# Autodesk Inventor assembly: 2022Drivetrain-v1
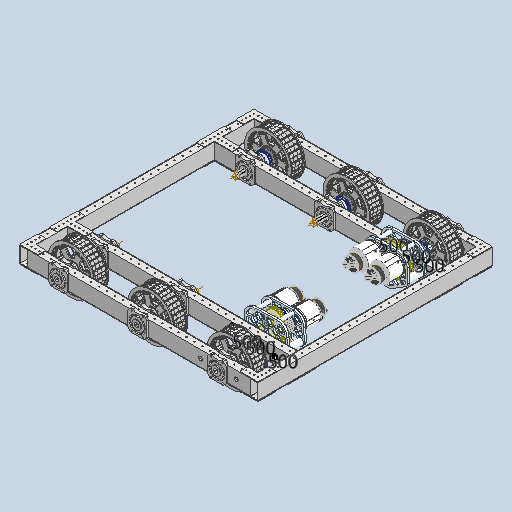
[picture p0: Inventor's stored thumbnail of the model, 512x512]
Saved by Autodesk Inventor 2022 (Build 260153000, 153)
## iProperties
Created: 2022-01-09
Part Number: 2022Drivetrain-v1
Document SubType Name: Assembly
Designer: merky
Author: merky
## Documents named in this file (11)
- C:\Users\tagaz\OneDrive\Documents\T3-Cad\CAD\2022 Parts\Drivetrain\2022Drivetrain-v1.iam
- C:\Users\tagaz\OneDrive\Documents\T3-Cad\CAD\2022 Parts\Generic\VersaFrame 28in.ipt
- C:\Users\tagaz\OneDrive\Documents\T3-Cad\CAD\2022 Parts\Generic\VersaFrame 30in.ipt
- C:\Users\tagaz\OneDrive\Documents\T3-Cad\CAD\VersaBlock Assembly.iam
- C:\Users\tagaz\OneDrive\Documents\T3-Cad\CAD\2022 Parts\Generic\VersaBlock Assemblyv2.iam
- C:\Users\tagaz\OneDrive\Documents\T3-Cad\CAD\Traction Wheel Assembly.iam
- C:\Users\tagaz\OneDrive\Documents\T3-Cad\CAD\6in x 1.5in Wheel.iam
- C:\Users\tagaz\OneDrive\Documents\T3-Cad\CAD\Generic and Stock\T Gusset.ipt
- C:\Users\tagaz\OneDrive\Documents\T3-Cad\CAD\2022 Parts\Generic\ShortenedVersaGusset 90o.ipt
- C:\Users\tagaz\OneDrive\Documents\T3-Cad\CAD\Generic and Stock\15T Sprocket.ipt
- C:\Users\tagaz\OneDrive\Documents\T3-Cad\CAD\2022 Parts\Generic\NewGearboxAssembly.iam
## Components (40 placed, 10 different names)
1. 15T Sprocket:1 — Insert:11
2. 15T Sprocket:2 — Insert:12
3. VersaFrame 28in:4 — Mate:17, Flush:9, Flush:10, Mate:27, Mate:28, Mate:30, Mate:31, Mate:33, Mate:34, Flush:11, Flush:13, Flush:16, Flush:18
4. VersaFrame 28in:3 — Mate:16, Flush:7, Flush:8, Mate:18, Mate:19, Mate:21, Mate:22, Mate:24, Mate:25, Flush:19, Flush:21, Flush:24, Flush:26
5. VersaFrame 30in:2 — Flush:1, Flush:2, Mate:1, Flush:3, Flush:4, Mate:3, Flush:5, Flush:6, Mate:6, Mate:9, Mate:12, Mate:15, Mate:16, Flush:7, Flush:8, Mate:17, Flush:9, Flush:10, Mate:20, Mate:23, Mate:26, Mate:29, Mate:32, Mate:35, Mate:36, Flush:12, Mate:37, Flush:14, Mate:40, Flush:20, Mate:41, Flush:22, Mate:48, Flush:35, Mate:49, Flush:37, Mate:50, Flush:40, Mate:51, Flush:42
6. VersaFrame 30in:1 — Flush:1, Flush:2, Mate:2, Mate:38, Flush:15, Mate:39, Flush:17, Mate:42, Flush:23, Mate:43, Flush:25, Mate:46, Flush:31, Mate:47, Flush:34
7. VersaFrame 28in:2 — Mate:3, Flush:5, Flush:6, Mate:10, Mate:11, Mate:13, Mate:14, Flush:32, Flush:39, Flush:41, Insert:8
8. VersaFrame 28in:1 — Mate:1, Flush:3, Flush:4, Mate:2, Mate:4, Mate:5, Mate:7, Mate:8, Flush:33, Flush:36, Flush:38, Insert:7
9. NewGearboxAssembly:1 [sub-assembly] — Insert:7, Insert:9, Insert:12
10. VersaBlock Assembly:1 [sub-assembly] — Mate:10, Mate:11, Mate:12, Insert:6
11. VersaBlock Assembly:3 [sub-assembly] — Mate:7, Mate:8, Mate:9, Insert:4
12. VersaBlock Assembly:4 [sub-assembly] — Mate:4, Mate:5, Mate:6, Insert:3
13. VersaBlock Assemblyv2:1 [sub-assembly] — Mate:13, Mate:14, Mate:15, Insert:5
14. Traction Wheel Assembly:1 [sub-assembly] — Insert:3
15. Traction Wheel Assembly:2 [sub-assembly] — Insert:4
16. Traction Wheel Assembly:3 [sub-assembly] — Insert:5
17. Traction Wheel Assembly:4 [sub-assembly] — Insert:6
18. 6in x 1.5in Wheel:1 [sub-assembly] — Insert:10
19. 6in x 1.5in Wheel:2 [sub-assembly] — Insert:9
20. VersaBlock Assembly:5 [sub-assembly] — Mate:18, Mate:19, Mate:20
21. VersaBlock Assembly:6 [sub-assembly] — Mate:21, Mate:22, Mate:23
22. VersaBlock Assembly:7 [sub-assembly] — Mate:24, Mate:25, Mate:26
23. VersaBlock Assembly:8 [sub-assembly] — Mate:33, Mate:34, Mate:35
24. VersaBlock Assembly:9 [sub-assembly] — Mate:30, Mate:31, Mate:32
25. VersaBlock Assembly:10 [sub-assembly] — Mate:27, Mate:28, Mate:29
26. NewGearboxAssembly:2 [sub-assembly] — Insert:8, Insert:10, Insert:11
27. T Gusset:1 — Mate:48, Flush:35, Flush:36
28. T Gusset:2 — Mate:49, Flush:37, Flush:38
29. T Gusset:5 — Mate:46, Flush:31, Flush:32
30. T Gusset:6 — Mate:47, Flush:33, Flush:34
31. T Gusset:7 — Mate:51, Flush:41, Flush:42
32. T Gusset:8 — Mate:50, Flush:39, Flush:40
33. ShortenedVersaGusset 90o:1 — Mate:40, Flush:19, Flush:20
34. ShortenedVersaGusset 90o:2 — Mate:41, Flush:21, Flush:22
35. ShortenedVersaGusset 90o:3 — Mate:37, Flush:13, Flush:14
36. ShortenedVersaGusset 90o:4 — Mate:36, Flush:11, Flush:12
37. ShortenedVersaGusset 90o:5 — Mate:39, Flush:17, Flush:18
38. ShortenedVersaGusset 90o:6 — Mate:38, Flush:15, Flush:16
39. ShortenedVersaGusset 90o:7 — Mate:43, Flush:25, Flush:26
40. ShortenedVersaGusset 90o:8 — Mate:42, Flush:23, Flush:24
## Relationships (97: Mate 49, Flush 38, Insert 10)
- Flush:1: VersaFrame 30in:2 ↔ VersaFrame 30in:1
- Flush:2: VersaFrame 30in:2 ↔ VersaFrame 30in:1
- Mate:1: VersaFrame 30in:2 ↔ VersaFrame 28in:1
- Flush:3: VersaFrame 30in:2 ↔ VersaFrame 28in:1
- Flush:4 (127 mm): VersaFrame 30in:2 ↔ VersaFrame 28in:1
- Mate:2: VersaFrame 30in:1 ↔ VersaFrame 28in:1
- Mate:3: VersaFrame 30in:2 ↔ VersaFrame 28in:2
- Flush:5: VersaFrame 30in:2 ↔ VersaFrame 28in:2
- Flush:6 (127 mm): VersaFrame 30in:2 ↔ VersaFrame 28in:2
- Mate:4: VersaFrame 28in:1 ↔ VersaBlock Assembly:4
- Mate:5: VersaFrame 28in:1 ↔ VersaBlock Assembly:4
- Mate:6 (71.0692 mm): VersaFrame 30in:2 ↔ VersaBlock Assembly:4
- Mate:7: VersaFrame 28in:1 ↔ VersaBlock Assembly:3
- Mate:8: VersaFrame 28in:1 ↔ VersaBlock Assembly:3
- Mate:9 (325.0692 mm): VersaFrame 30in:2 ↔ VersaBlock Assembly:3
- Mate:10: VersaFrame 28in:2 ↔ VersaBlock Assembly:1
- Mate:11: VersaFrame 28in:2 ↔ VersaBlock Assembly:1
- Mate:12 (71.0692 mm): VersaFrame 30in:2 ↔ VersaBlock Assembly:1
- Mate:13: VersaFrame 28in:2 ↔ VersaBlock Assemblyv2:1
- Mate:14: VersaFrame 28in:2 ↔ VersaBlock Assemblyv2:1
- Mate:15 (325.0692 mm): VersaFrame 30in:2 ↔ VersaBlock Assemblyv2:1
- Insert:3 (-63.5 mm): VersaBlock Assembly:4 ↔ Traction Wheel Assembly:1
- Insert:4 (-63.5 mm): VersaBlock Assembly:3 ↔ Traction Wheel Assembly:2
- Mate:16: VersaFrame 28in:3 ↔ VersaFrame 30in:2
- Flush:7: VersaFrame 28in:3 ↔ VersaFrame 30in:2
- Flush:8: VersaFrame 28in:3 ↔ VersaFrame 30in:2
- Mate:17: VersaFrame 28in:4 ↔ VersaFrame 30in:2
- Flush:9: VersaFrame 28in:4 ↔ VersaFrame 30in:2
- Flush:10: VersaFrame 28in:4 ↔ VersaFrame 30in:2
- Insert:5 (-63.5 mm): VersaBlock Assemblyv2:1 ↔ Traction Wheel Assembly:3
- Insert:6 (-63.5 mm): VersaBlock Assembly:1 ↔ Traction Wheel Assembly:4
- Mate:18: VersaFrame 28in:3 ↔ VersaBlock Assembly:5
- Mate:19: VersaFrame 28in:3 ↔ VersaBlock Assembly:5
- Mate:20 (71.0692 mm): VersaFrame 30in:2 ↔ VersaBlock Assembly:5
- Mate:21: VersaFrame 28in:3 ↔ VersaBlock Assembly:6
- Mate:22: VersaFrame 28in:3 ↔ VersaBlock Assembly:6
- Mate:23 (325.0692 mm): VersaFrame 30in:2 ↔ VersaBlock Assembly:6
- Mate:24: VersaFrame 28in:3 ↔ VersaBlock Assembly:7
- Mate:25: VersaFrame 28in:3 ↔ VersaBlock Assembly:7
- Mate:26 (579.0692 mm): VersaFrame 30in:2 ↔ VersaBlock Assembly:7
- Mate:27: VersaFrame 28in:4 ↔ VersaBlock Assembly:10
- Mate:28: VersaFrame 28in:4 ↔ VersaBlock Assembly:10
- Mate:29 (579.0692 mm): VersaFrame 30in:2 ↔ VersaBlock Assembly:10
- Mate:30: VersaFrame 28in:4 ↔ VersaBlock Assembly:9
- Mate:31: VersaFrame 28in:4 ↔ VersaBlock Assembly:9
- Mate:32 (325.0692 mm): VersaFrame 30in:2 ↔ VersaBlock Assembly:9
- Mate:33: VersaFrame 28in:4 ↔ VersaBlock Assembly:8
- Mate:34: VersaFrame 28in:4 ↔ VersaBlock Assembly:8
- Mate:35 (71.0692 mm): VersaFrame 30in:2 ↔ VersaBlock Assembly:8
- Mate:36: VersaFrame 30in:2 ↔ ShortenedVersaGusset 90o:4
- Flush:11: VersaFrame 28in:4 ↔ ShortenedVersaGusset 90o:4
- Flush:12: VersaFrame 30in:2 ↔ ShortenedVersaGusset 90o:4
- Mate:37: VersaFrame 30in:2 ↔ ShortenedVersaGusset 90o:3
- Flush:13: VersaFrame 28in:4 ↔ ShortenedVersaGusset 90o:3
- Flush:14: VersaFrame 30in:2 ↔ ShortenedVersaGusset 90o:3
- Mate:38: VersaFrame 30in:1 ↔ ShortenedVersaGusset 90o:6
- Flush:15: VersaFrame 30in:1 ↔ ShortenedVersaGusset 90o:6
- Flush:16: VersaFrame 28in:4 ↔ ShortenedVersaGusset 90o:6
- Mate:39: VersaFrame 30in:1 ↔ ShortenedVersaGusset 90o:5
- Flush:17: VersaFrame 30in:1 ↔ ShortenedVersaGusset 90o:5
- Flush:18: VersaFrame 28in:4 ↔ ShortenedVersaGusset 90o:5
- Mate:40: VersaFrame 30in:2 ↔ ShortenedVersaGusset 90o:1
- Flush:19: VersaFrame 28in:3 ↔ ShortenedVersaGusset 90o:1
- Flush:20: VersaFrame 30in:2 ↔ ShortenedVersaGusset 90o:1
- Mate:41: VersaFrame 30in:2 ↔ ShortenedVersaGusset 90o:2
- Flush:21: VersaFrame 28in:3 ↔ ShortenedVersaGusset 90o:2
- Flush:22: VersaFrame 30in:2 ↔ ShortenedVersaGusset 90o:2
- Mate:42: VersaFrame 30in:1 ↔ ShortenedVersaGusset 90o:8
- Flush:23: VersaFrame 30in:1 ↔ ShortenedVersaGusset 90o:8
- Flush:24: VersaFrame 28in:3 ↔ ShortenedVersaGusset 90o:8
- Mate:43: VersaFrame 30in:1 ↔ ShortenedVersaGusset 90o:7
- Flush:25: VersaFrame 30in:1 ↔ ShortenedVersaGusset 90o:7
- Flush:26: VersaFrame 28in:3 ↔ ShortenedVersaGusset 90o:7
- Mate:46: VersaFrame 30in:1 ↔ T Gusset:5
- Flush:31: VersaFrame 30in:1 ↔ T Gusset:5
- Flush:32: VersaFrame 28in:2 ↔ T Gusset:5
- Mate:47: VersaFrame 30in:1 ↔ T Gusset:6
- Flush:33: VersaFrame 28in:1 ↔ T Gusset:6
- Flush:34: VersaFrame 30in:1 ↔ T Gusset:6
- Mate:48: VersaFrame 30in:2 ↔ T Gusset:1
- Flush:35: VersaFrame 30in:2 ↔ T Gusset:1
- Flush:36: VersaFrame 28in:1 ↔ T Gusset:1
- Mate:49: VersaFrame 30in:2 ↔ T Gusset:2
- Flush:37: VersaFrame 30in:2 ↔ T Gusset:2
- Flush:38: VersaFrame 28in:1 ↔ T Gusset:2
- Mate:50: VersaFrame 30in:2 ↔ T Gusset:8
- Flush:39: VersaFrame 28in:2 ↔ T Gusset:8
- Flush:40: VersaFrame 30in:2 ↔ T Gusset:8
- Mate:51: VersaFrame 30in:2 ↔ T Gusset:7
- Flush:41: VersaFrame 28in:2 ↔ T Gusset:7
- Flush:42: VersaFrame 30in:2 ↔ T Gusset:7
- Insert:7: VersaFrame 28in:1 ↔ NewGearboxAssembly:1
- Insert:8: VersaFrame 28in:2 ↔ NewGearboxAssembly:2
- Insert:9 (-10.16 mm): NewGearboxAssembly:1 ↔ 6in x 1.5in Wheel:2
- Insert:10 (-10.16 mm): 6in x 1.5in Wheel:1 ↔ NewGearboxAssembly:2
- Insert:11 (19.05 mm): 15T Sprocket:1 ↔ NewGearboxAssembly:2
- Insert:12 (12.7 mm): 15T Sprocket:2 ↔ NewGearboxAssembly:1
